# Autodesk Inventor assembly: front_rear_unit_assembly_fixed
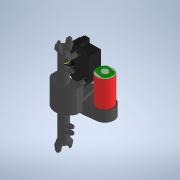
[picture p0: Inventor's stored thumbnail of the model, 180x180]
Saved by Autodesk Inventor 2020 (Build 240168000, 168)
## iProperties
Created: 2019-12-06
Part Number: front_rear_unit_assembly_fixed
Document SubType Name: Assembly
Designer: maste
Author: maste
## Documents named in this file (8)
- C:\Users\maste\Documents\GitHub\autobot\robot_model\front_rear_unit_assembly_fixed.iam
- C:\Users\maste\Documents\GitHub\autobot\robot_model\RCT-P004_front_rear_axle_simplified.ipt
- C:\Users\maste\Documents\GitHub\autobot\robot_model\RCT-H111_upper_link_mount.ipt
- C:\Users\maste\Documents\GitHub\autobot\robot_model\servo_plate_assembly.iam
- C:\Users\maste\Documents\GitHub\autobot\robot_model\E600T_RC390_motor_front.ipt
- C:\Users\maste\Documents\GitHub\autobot\robot_model\H016 (2).ipt
- C:\Users\maste\Documents\GitHub\autobot\robot_model\RCT-H022_washer_25_55_05.ipt
- C:\Users\maste\Documents\GitHub\autobot\robot_model\H016.ipt
## Components (7 placed, 7 different names)
1. RCT-P004_front_rear_axle_simplified:1 — Mate:1, Mate:2, Mate:3, Mate:4, Mate:5, Mate:6, Mate:7, Mate:8
2. RCT-H111_upper_link_mount:1 — Mate:1, Mate:2, Mate:3, Mate:9, Mate:10, Mate:11, Mate:12, Mate:13
3. servo_plate_assembly:1 [sub-assembly] — Mate:4, Mate:5, Mate:6
4. E600T_RC390_motor_front:1 — Mate:7, Mate:8
5. H016 (2):1 — Mate:9, Mate:10
6. RCT-H022_washer_25_55_05:1 — Mate:11, Mate:12, Mate:14
7. H016:1 — Mate:13, Mate:14
## Relationships (14: Mate 14)
- Mate:1: RCT-P004_front_rear_axle_simplified:1 ↔ RCT-H111_upper_link_mount:1
- Mate:2: RCT-P004_front_rear_axle_simplified:1 ↔ RCT-H111_upper_link_mount:1
- Mate:3: RCT-P004_front_rear_axle_simplified:1 ↔ RCT-H111_upper_link_mount:1
- Mate:4: RCT-P004_front_rear_axle_simplified:1 ↔ servo_plate_assembly:1
- Mate:5: RCT-P004_front_rear_axle_simplified:1 ↔ servo_plate_assembly:1
- Mate:6: RCT-P004_front_rear_axle_simplified:1 ↔ servo_plate_assembly:1
- Mate:7: RCT-P004_front_rear_axle_simplified:1 ↔ E600T_RC390_motor_front:1
- Mate:8: RCT-P004_front_rear_axle_simplified:1 ↔ E600T_RC390_motor_front:1
- Mate:9: RCT-H111_upper_link_mount:1 ↔ H016 (2):1
- Mate:10: RCT-H111_upper_link_mount:1 ↔ H016 (2):1
- Mate:11: RCT-H111_upper_link_mount:1 ↔ RCT-H022_washer_25_55_05:1
- Mate:12: RCT-H111_upper_link_mount:1 ↔ RCT-H022_washer_25_55_05:1
- Mate:13: RCT-H111_upper_link_mount:1 ↔ H016:1
- Mate:14: RCT-H022_washer_25_55_05:1 ↔ H016:1
